# Autodesk Inventor assembly: ESTOP V2 PCB
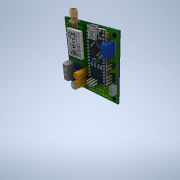
[picture p0: Inventor's stored thumbnail of the model, 180x180]
Saved by Autodesk Inventor 2021 (Build 250183000, 183)
## iProperties
Created: 2019-10-02
Part Number: ESTOP V2 PCB
Document SubType Name: Assembly
Designer: rybit
Author: rybit
## Documents named in this file (11)
- G:\Box Sync\Eagle\Projects\E Stop v2\ESTOP V2\ESTOP V2 PCB.iam
- G:\Box Sync\Eagle\Projects\E Stop v2\ESTOP V2\arduino nano.iam
- G:\Box Sync\Eagle\Projects\E Stop v2\ESTOP V2\estop v2.iam
- G:\Box Sync\Eagle\Projects\E Stop v2\ESTOP V2\Trimpot_3296W.ipt
- G:\Box Sync\Eagle\Projects\E Stop v2\ESTOP V2\Terminal-Screw-3A-3way.ipt
- G:\Box Sync\Eagle\Projects\E Stop v2\ESTOP V2\LED RGB 8mm.ipt
- G:\Box Sync\Eagle\Projects\E Stop v2\ESTOP V2\pin header.iam
- G:\Box Sync\Eagle\Projects\E Stop v2\ESTOP V2\1.5mm JST.ipt
- G:\Box Sync\Eagle\Projects\E Stop v2\ESTOP V2\capacitor.iam
- G:\Box Sync\Eagle\Projects\E Stop v2\ESTOP V2\res0805.ipt
- G:\Box Sync\Eagle\Projects\E Stop v2\ESTOP V2\DD0503MA ULTRA MINI DC 3.7V 4.5V 5V TO 3.3V DC DC STEP DOWN CONVERTER BUCK MODULE.iam
## Components (22 placed, 10 different names)
1. arduino nano:1 [sub-assembly] — Angle:1, Insert:1
2. estop v2.brd:1 [sub-assembly] — Angle:1, Insert:1, Insert:2, Angle:2, Insert:3, Angle:3, Mate:1, Angle:4, Tangent:1, Tangent:2, Mate:5, Flush:7, Flush:8, Mate:6, Flush:9, Flush:10, Insert:4, Angle:5, Insert:5, Insert:6, Angle:6, Angle:7, Mate:7, Mate:8, Mate:9, Mate:10, Mate:11, Angle:8, Angle:9, Angle:10, Angle:11, Angle:12, Flush:11, Flush:12, Flush:13, Flush:14, Flush:15, Flush:16, Flush:17, Flush:18, Flush:19, Flush:20, Mate:15, Flush:27, Flush:28
3. Trimpot_3296W:1 — Insert:2, Angle:2
4. Terminal-Screw-3A-3way:1 — Insert:3, Angle:3
5. LED RGB 8mm:1 — Mate:1, Angle:4, Tangent:1, Tangent:2
6. pin header:1 [sub-assembly] — Mate:2, Flush:1, Flush:2, Mate:5, Flush:7
7. pin header:2 [sub-assembly] — Mate:2, Flush:1, Flush:2, Flush:8
8. pin header:3 [sub-assembly] — Mate:3, Flush:3, Flush:4, Mate:6
9. pin header:4 [sub-assembly] — Mate:3, Flush:3, Flush:4, Mate:4, Flush:5, Flush:6, Flush:9
10. pin header:5 [sub-assembly] — Mate:4, Flush:5, Flush:6, Flush:10
11. 1.5mm JST:1 — Insert:4, Angle:5
12. capacitor:1 [sub-assembly] — Insert:6, Angle:6
13. capacitor:2 [sub-assembly] — Insert:5, Angle:7
14. res0805:1 — Mate:7, Angle:12, Flush:15, Flush:20
15. res0805:2 — Mate:8, Angle:11, Flush:14, Flush:19
16. res0805:3 — Mate:9, Angle:10, Flush:13, Flush:18
17. res0805:4 — Mate:10, Angle:9, Flush:12, Flush:17
18. res0805:5 — Mate:11, Angle:8, Flush:11, Flush:16
19. DD0503MA ULTRA MINI DC 3.7V 4.5V 5V TO 3.3V DC DC STEP DOWN CONVERTER BUCK MODULE:1 [sub-assembly] — Mate:14, Flush:25, Flush:26, Flush:27, Flush:28
20. pin header:6 [sub-assembly] — Mate:15
21. pin header:7 [sub-assembly] — Flush:25
22. pin header:8 [sub-assembly] — Mate:14, Flush:26
## Relationships (63: Flush 28, Mate 15, Angle 12, Insert 6, Tangent 2)
- Angle:1 (0 deg): arduino nano:1 ↔ estop v2.brd:1
- Insert:1 (2.5 mm): arduino nano:1 ↔ estop v2.brd:1
- Insert:2 (0.381 mm): estop v2.brd:1 ↔ Trimpot_3296W:1
- Angle:2 (0 deg): estop v2.brd:1 ↔ Trimpot_3296W:1
- Insert:3 (0.508 mm): estop v2.brd:1 ↔ Terminal-Screw-3A-3way:1
- Angle:3 (0 deg): estop v2.brd:1 ↔ Terminal-Screw-3A-3way:1
- Mate:1: estop v2.brd:1 ↔ LED RGB 8mm:1
- Angle:4 (0 deg): estop v2.brd:1 ↔ LED RGB 8mm:1
- Tangent:1: estop v2.brd:1 ↔ LED RGB 8mm:1
- Tangent:2 (9.05 mm): estop v2.brd:1 ↔ LED RGB 8mm:1
- Mate:2: pin header:1 ↔ pin header:2
- Flush:1: pin header:1 ↔ pin header:2
- Flush:2: pin header:1 ↔ pin header:2
- Mate:3: pin header:3 ↔ pin header:4
- Flush:3: pin header:3 ↔ pin header:4
- Flush:4: pin header:3 ↔ pin header:4
- Mate:4: pin header:4 ↔ pin header:5
- Flush:5: pin header:4 ↔ pin header:5
- Flush:6: pin header:4 ↔ pin header:5
- Mate:5: estop v2.brd:1 ↔ pin header:1
- Flush:7 (2.54 mm): estop v2.brd:1 ↔ pin header:1
- Flush:8 (22.86 mm): estop v2.brd:1 ↔ pin header:2
- Mate:6: estop v2.brd:1 ↔ pin header:3
- Flush:9 (2.54 mm): estop v2.brd:1 ↔ pin header:4
- Flush:10 (31.75 mm): estop v2.brd:1 ↔ pin header:5
- Insert:4: estop v2.brd:1 ↔ 1.5mm JST:1
- Angle:5 (0 deg): estop v2.brd:1 ↔ 1.5mm JST:1
- Insert:5: estop v2.brd:1 ↔ capacitor:2
- Insert:6: estop v2.brd:1 ↔ capacitor:1
- Angle:6 (0 deg): estop v2.brd:1 ↔ capacitor:1
- Angle:7 (0 deg): estop v2.brd:1 ↔ capacitor:2
- Mate:7: estop v2.brd:1 ↔ res0805:1
- Mate:8: estop v2.brd:1 ↔ res0805:2
- Mate:9: estop v2.brd:1 ↔ res0805:3
- Mate:10: estop v2.brd:1 ↔ res0805:4
- Mate:11: estop v2.brd:1 ↔ res0805:5
- Angle:8 (0 deg): estop v2.brd:1 ↔ res0805:5
- Angle:9 (0 deg): estop v2.brd:1 ↔ res0805:4
- Angle:10 (0 deg): estop v2.brd:1 ↔ res0805:3
- Angle:11 (0 deg): estop v2.brd:1 ↔ res0805:2
- Angle:12 (0 deg): estop v2.brd:1 ↔ res0805:1
- Flush:11 (-8.89 mm): estop v2.brd:1 ↔ res0805:5
- Flush:12 (-8.89 mm): estop v2.brd:1 ↔ res0805:4
- Flush:13 (-8.89 mm): estop v2.brd:1 ↔ res0805:3
- Flush:14 (-8.89 mm): estop v2.brd:1 ↔ res0805:2
- Flush:15 (-8.89 mm): estop v2.brd:1 ↔ res0805:1
- Flush:16 (-10.033 mm): estop v2.brd:1 ↔ res0805:5
- Flush:17 (-13.8557 mm): estop v2.brd:1 ↔ res0805:4
- Flush:18 (-17.6657 mm): estop v2.brd:1 ↔ res0805:3
- Flush:19 (-21.4757 mm): estop v2.brd:1 ↔ res0805:2
- Flush:20 (-25.2857 mm): estop v2.brd:1 ↔ res0805:1
- [Mate]: pin header:6 ↔ pin header:7
- [Flush]: pin header:6 ↔ pin header:7
- [Flush]: pin header:6 ↔ pin header:7
- [Mate]: pin header:7 ↔ pin header:8
- [Flush]: pin header:7 ↔ pin header:8
- [Flush]: pin header:7 ↔ pin header:8
- Mate:14: DD0503MA ULTRA MINI DC 3.7V 4.5V 5V TO 3.3V DC DC STEP DOWN CONVERTER BUCK MODULE:1 ↔ pin header:8
- Flush:25: DD0503MA ULTRA MINI DC 3.7V 4.5V 5V TO 3.3V DC DC STEP DOWN CONVERTER BUCK MODULE:1 ↔ pin header:7
- Flush:26 (-0.0508 mm): DD0503MA ULTRA MINI DC 3.7V 4.5V 5V TO 3.3V DC DC STEP DOWN CONVERTER BUCK MODULE:1 ↔ pin header:8
- Mate:15: estop v2.brd:1 ↔ pin header:6
- Flush:27 (10.16 mm): estop v2.brd:1 ↔ DD0503MA ULTRA MINI DC 3.7V 4.5V 5V TO 3.3V DC DC STEP DOWN CONVERTER BUCK MODULE:1
- Flush:28 (11.4808 mm): estop v2.brd:1 ↔ DD0503MA ULTRA MINI DC 3.7V 4.5V 5V TO 3.3V DC DC STEP DOWN CONVERTER BUCK MODULE:1
## Named parameters: d52_d14 = 0 mm, d53_d15 = 0 mm, d54_d16 = 0 mm, d55_d17 = 0 mm, d56_d18 = 0 mm, d57_d19 = 0 mm
